# Autodesk Inventor assembly: OwnSpectr_TubeHolder
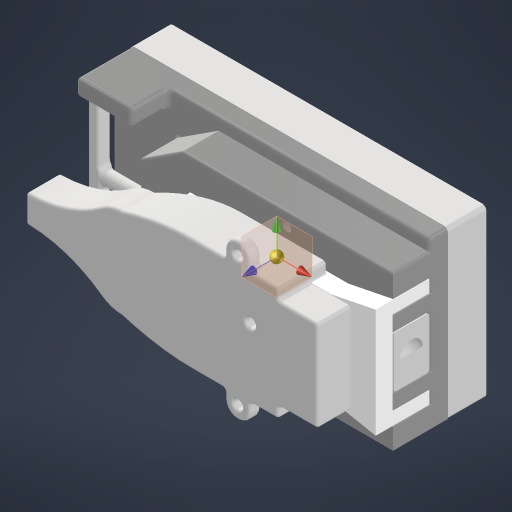
[picture p0: Inventor's stored thumbnail of the model, 512x512]
Saved by Autodesk Inventor 2024.1 (Build 281209000, 209)
## iProperties
Created: 2024-08-12
Part Number: OwnSpectr_TubeHolder
Document SubType Name: Assembly
Designer: Tim Jäger
Author: Tim Jäger
## Documents named in this file (8)
- D:\Users\Tim\VUB\Master_Embedded\Master_Thesis\Files3D\OwnSpectr_TubeHolder.iam
- D:\Users\Tim\VUB\Master_Embedded\Master_Thesis\Files3D\OwnSpectr_TubeHolder.ipt
- D:\Users\Tim\VUB\Master_Embedded\Master_Thesis\Files3D\OwnSpectr_TubeHolder_B.ipt
- D:\Users\Tim\VUB\Master_Embedded\Master_Thesis\Files3D\OwnSpectr_TubeHolder_C.ipt
- D:\Users\Tim\VUB\Master_Embedded\Master_Thesis\Files3D\OwnSpectr_TubeHolder_D.ipt
- D:\Users\Tim\VUB\Master_Embedded\Master_Thesis\Files3D\Cuvette.iam
- D:\Users\Tim\VUB\Master_Embedded\Master_Thesis\Files3D\OwnSpectr_TubeHolder_E.ipt
- D:\Users\Tim\VUB\Master_Embedded\Master_Thesis\Files3D\OwnSpectr_TubeHolder_F.ipt
## Components (7 placed, 7 different names)
1. OwnSpectr_TubeHolder:1 — Mate:1, Mate:2, Mate:3, Flush:1, Mate:4, Angle:1, Mate:5, Flush:2, Angle:7, Mate:7, Mate:9, Mate:10, Mate:11, Angle:8
2. OwnSpectr_TubeHolder_B:1 — Mate:1, Mate:2, Mate:3, Mate:12, Mate:13, Angle:9
3. OwnSpectr_TubeHolder_C:1 — Flush:1, Mate:4, Angle:1, Mate:5, Mate:6, Mate:8
4. OwnSpectr_TubeHolder_D:1 — Flush:2, Angle:7, Mate:6
5. Cuvette:1 [sub-assembly] — Mate:7, Mate:8, Mate:9
6. OwnSpectr_TubeHolder_E:1 — Mate:10, Mate:11, Angle:8
7. OwnSpectr_TubeHolder_F:1 — Mate:12, Mate:13, Angle:9
## Relationships (19: Mate 13, Angle 4, Flush 2)
- Mate:1: OwnSpectr_TubeHolder:1 ↔ OwnSpectr_TubeHolder_B:1
- Mate:2 (0.18 mm): OwnSpectr_TubeHolder:1 ↔ OwnSpectr_TubeHolder_B:1
- Mate:3 (0.36 mm): OwnSpectr_TubeHolder:1 ↔ OwnSpectr_TubeHolder_B:1
- Flush:1: OwnSpectr_TubeHolder:1 ↔ OwnSpectr_TubeHolder_C:1
- Mate:4: OwnSpectr_TubeHolder:1 ↔ OwnSpectr_TubeHolder_C:1
- Angle:1 (0 deg): OwnSpectr_TubeHolder:1 ↔ OwnSpectr_TubeHolder_C:1
- Mate:5: OwnSpectr_TubeHolder:1 ↔ OwnSpectr_TubeHolder_C:1
- Flush:2: OwnSpectr_TubeHolder:1 ↔ OwnSpectr_TubeHolder_D:1
- Angle:7 (0 deg): OwnSpectr_TubeHolder:1 ↔ OwnSpectr_TubeHolder_D:1
- Mate:6: OwnSpectr_TubeHolder_C:1 ↔ OwnSpectr_TubeHolder_D:1
- Mate:7 (0.5 mm): OwnSpectr_TubeHolder:1 ↔ Cuvette:1
- Mate:8: OwnSpectr_TubeHolder_C:1 ↔ Cuvette:1
- Mate:9: OwnSpectr_TubeHolder:1 ↔ Cuvette:1
- Mate:10: OwnSpectr_TubeHolder:1 ↔ OwnSpectr_TubeHolder_E:1
- Mate:11: OwnSpectr_TubeHolder:1 ↔ OwnSpectr_TubeHolder_E:1
- Angle:8 (0 deg): OwnSpectr_TubeHolder:1 ↔ OwnSpectr_TubeHolder_E:1
- Mate:12: OwnSpectr_TubeHolder_B:1 ↔ OwnSpectr_TubeHolder_F:1
- Mate:13: OwnSpectr_TubeHolder_B:1 ↔ OwnSpectr_TubeHolder_F:1
- Angle:9 (0 deg): OwnSpectr_TubeHolder_B:1 ↔ OwnSpectr_TubeHolder_F:1
